# Autodesk Inventor assembly: FinalCarro
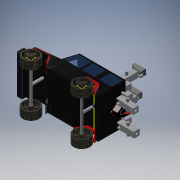
[picture p0: Inventor's stored thumbnail of the model, 180x180]
Saved by Autodesk Inventor 2017 (Build 210142000, 142)
## iProperties
Part Number: FinalCarro
Material: Genérico
Document SubType Name: Assembly
Designer: Ghost
Author: Ghost
## Documents named in this file (9)
- C:\Users\Ghost\Desktop\UVG Semestre 8\Dibujo Mecanico\ProyectoTransformer\FinalCarro.iam
- C:\Users\Ghost\Desktop\UVG Semestre 8\Dibujo Mecanico\ProyectoTransformer\ProyectoTransformer\Bumper.ipt
- C:\Users\Ghost\Desktop\UVG Semestre 8\Dibujo Mecanico\ProyectoTransformer\ProyectoTransformer\CabezaCarro.ipt
- C:\Users\Ghost\Desktop\UVG Semestre 8\Dibujo Mecanico\ProyectoTransformer\ProyectoTransformer\PuertaMarco.iam
- C:\Users\Ghost\Desktop\UVG Semestre 8\Dibujo Mecanico\ProyectoTransformer\ProyectoTransformer\llanta.ipt
- C:\Users\Ghost\Desktop\UVG Semestre 8\Dibujo Mecanico\ProyectoTransformer\ProyectoTransformer\Hombro.ipt
- C:\Users\Ghost\Desktop\UVG Semestre 8\Dibujo Mecanico\ProyectoTransformer\ProyectoTransformer\Union pie.ipt
- C:\Users\Ghost\Desktop\UVG Semestre 8\Dibujo Mecanico\ProyectoTransformer\ProyectoTransformer\Ante pierna.ipt
- C:\Users\Ghost\Desktop\UVG Semestre 8\Dibujo Mecanico\ProyectoTransformer\ProyectoTransformer\Pie.ipt
## Components (23 placed, 8 different names)
1. Bumper:1 — Insertar:1, Insertar:2, Insertar:5, Insertar:6
2. CabezaCarro:1 — Coincidencia:1, Insertar:3
3. PuertaMarco:1 [sub-assembly] — Insertar:1, Insertar:2, Coincidencia:1, Insertar:3, Insertar:4, Insertar:7, Insertar:9, Insertar:10, Insertar:18, Insertar:19
4. llanta:1 — Insertar:5
5. llanta:2 — Insertar:6
6. llanta:3 — Insertar:7
7. llanta:4 — Insertar:4
8. Hombro:1 — Insertar:16, Insertar:19
9. Hombro:2 — Insertar:9, Insertar:12
10. Hombro:3 — Insertar:17, Insertar:18
11. Hombro:4 — Insertar:10, Insertar:20
12. Union pie:1 — Insertar:16, Coincidencia:2, Coincidencia:3
13. Union pie:2 — Insertar:17, Coincidencia:4, Coincidencia:5
14. Union pie:4 — Insertar:12, Coincidencia:8, Coincidencia:9
15. Ante pierna:1 — Coincidencia:8, Coincidencia:9, Insertar:22
16. Ante pierna:2 — Coincidencia:4, Coincidencia:5
17. Ante pierna:4 — Coincidencia:2, Coincidencia:3
18. Union pie:5 — Coincidencia:10, Coincidencia:11, Insertar:20
19. Ante pierna:6 — Coincidencia:10, Coincidencia:11, Insertar:21
20. Union pie:6 — Insertar:21, Coincidencia:14, Coincidencia:15
21. Union pie:7 — Insertar:22, Coincidencia:12, Coincidencia:13
22. Pie:1 — Coincidencia:12, Coincidencia:13
23. Pie:2 — Coincidencia:14, Coincidencia:15
## Relationships (30: Insert 17, Mate 13)
- Insertar:1: Bumper:1 ↔ PuertaMarco:1
- Insertar:2: Bumper:1 ↔ PuertaMarco:1
- Coincidencia:1 [Mate]: CabezaCarro:1 ↔ PuertaMarco:1
- Insertar:3: CabezaCarro:1 ↔ PuertaMarco:1
- Insertar:4: PuertaMarco:1 ↔ llanta:4
- Insertar:5: Bumper:1 ↔ llanta:1
- Insertar:6: Bumper:1 ↔ llanta:2
- Insertar:7: PuertaMarco:1 ↔ llanta:3
- Insertar:9: PuertaMarco:1 ↔ Hombro:2
- Insertar:10: PuertaMarco:1 ↔ Hombro:4
- Insertar:12: Hombro:2 ↔ Union pie:4
- Insertar:16: Hombro:1 ↔ Union pie:1
- Insertar:17: Hombro:3 ↔ Union pie:2
- Coincidencia:2 [Mate]: Union pie:1 ↔ Ante pierna:4
- Coincidencia:3 [Mate]: Union pie:1 ↔ Ante pierna:4
- Coincidencia:4 [Mate]: Union pie:2 ↔ Ante pierna:2
- Coincidencia:5 [Mate]: Union pie:2 ↔ Ante pierna:2
- Insertar:18: PuertaMarco:1 ↔ Hombro:3
- Insertar:19: PuertaMarco:1 ↔ Hombro:1
- Coincidencia:8 [Mate]: Union pie:4 ↔ Ante pierna:1
- Coincidencia:9 [Mate]: Union pie:4 ↔ Ante pierna:1
- Coincidencia:10 [Mate]: Union pie:5 ↔ Ante pierna:6
- Coincidencia:11 [Mate]: Union pie:5 ↔ Ante pierna:6
- Insertar:20: Hombro:4 ↔ Union pie:5
- Insertar:21: Ante pierna:6 ↔ Union pie:6
- Insertar:22: Ante pierna:1 ↔ Union pie:7
- Coincidencia:12 [Mate]: Union pie:7 ↔ Pie:1
- Coincidencia:13 [Mate]: Union pie:7 ↔ Pie:1
- Coincidencia:14 [Mate]: Union pie:6 ↔ Pie:2
- Coincidencia:15 [Mate]: Union pie:6 ↔ Pie:2
